# Autodesk Inventor assembly: Gripper Attempt 05
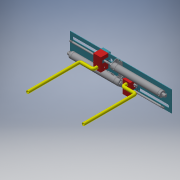
[picture p0: Inventor's stored thumbnail of the model, 180x180]
Saved by Autodesk Inventor 2016 (Build 200138000, 138)
## iProperties
Created: 2015-06-19
Part Number: Gripper Attempt 05
Document SubType Name: Assembly
Designer: steele
Mass: 1782.14 g
Surface Area: 5525.09 cm^2
Volume: 900.724 cm^3
Density: 1.97857 g/cm^3
Author: steele
## Documents named in this file (11)
- C:\snobotics\CAD-Development\robSteele\SnoBoticsSummer2015\Gripper\Gripper Attempt 05.iam
- C:\snobotics\CAD-MfgResources\McMaster-Carr\Air Cylinder\Pivot Mount Cylinders\Foot Bracket for 1_25 and 1_50 Bore\6498K340.ipt
- C:\snobotics\CAD-Development\robSteele\SnoBoticsSummer2015\Gripper\6498K681.ipt
- C:\snobotics\CAD-Development\robSteele\ipartComponents\Plate for Gripper.ipt
- C:\snobotics\CAD-Development\robSteele\SnoBoticsSummer2015\Gripper\Support For Arms.ipt
- C:\snobotics\CAD-Development\robSteele\SnoBoticsSummer2015\Gripper\Support Overlay on Gripper Side.ipt
- C:\snobotics\CAD-Development\robSteele\ipartComponents\ABS Arm.ipt
- C:\snobotics\CAD-MfgResources\McMaster-Carr\Quick Release Pin\94748A227.ipt
- C:\snobotics\autodesk\2015\FRC_FieldModel_2015\Parts\YELLOW_TOTE.ipt
- C:\snobotics\autodesk\2015\FRC_FieldModel_2015\Parts\RECYCLING_BIN_ASM.iam
- C:\snobotics\CAD-Development\robSteele\ipartComponents\Plate for Gripper\Plate for Gripper 5.5 x 27 x 1(_FS)8 x 3(_FS)8.ipt
## Components (16 placed, 9 different names)
1. Plate for Gripper 5.5 x 27 x 1(_FS)8 x 3(_FS)8:1 — Mate:1, Flush:1, Flush:2, Mate:2, Flush:3, Flush:4, Mate:9, Mate:13, Mate:14
2. 6498K340:1 — Mate:2, Flush:3, Flush:4, Mate:7
3. 6498K340:2 — Mate:1, Flush:1, Flush:2, Mate:8
4. 6498K681:1 — Mate:7
5. 6498K681:2 — Mate:8, Insert:3
6. Support For Arms:1 — Mate:9, Insert:3, Mate:10, Flush:10, Flush:13, Mate:12
7. Support For Arms:2 — Mate:13, Mate:14, Mate:15, Flush:14, Mate:16
8. Support Overlay on Gripper Side:1 — Mate:10, Flush:10, Flush:13, Mate:12, Insert:4, Insert:7
9. Support Overlay on Gripper Side:2 — Mate:15, Flush:14, Mate:16, Insert:6, Insert:8
10. ABS Arm:1 — Insert:4
11. ABS Arm:2 — Insert:6
12. 94748A227:1 — Insert:7
13. 94748A227:2 — Insert:8
14. YELLOW_TOTE:1
15. YELLOW_TOTE:2
16. RECYCLING_BIN_ASM:1 [sub-assembly]
## Relationships (23: Mate 11, Flush 7, Insert 5)
- Mate:1: Plate for Gripper 5.5 x 27 x 1(_FS)8 x 3(_FS)8:1 ↔ 6498K340:2
- Flush:1: Plate for Gripper 5.5 x 27 x 1(_FS)8 x 3(_FS)8:1 ↔ 6498K340:2
- Flush:2 (330.2 mm): Plate for Gripper 5.5 x 27 x 1(_FS)8 x 3(_FS)8:1 ↔ 6498K340:2
- Mate:2: Plate for Gripper 5.5 x 27 x 1(_FS)8 x 3(_FS)8:1 ↔ 6498K340:1
- Flush:3: Plate for Gripper 5.5 x 27 x 1(_FS)8 x 3(_FS)8:1 ↔ 6498K340:1
- Flush:4 (330.2 mm): Plate for Gripper 5.5 x 27 x 1(_FS)8 x 3(_FS)8:1 ↔ 6498K340:1
- Mate:7: 6498K340:1 ↔ 6498K681:1
- Mate:8: 6498K340:2 ↔ 6498K681:2
- Mate:9: Plate for Gripper 5.5 x 27 x 1(_FS)8 x 3(_FS)8:1 ↔ Support For Arms:1
- Insert:3: 6498K681:2 ↔ Support For Arms:1
- Mate:10: Support For Arms:1 ↔ Support Overlay on Gripper Side:1
- Flush:10: Support For Arms:1 ↔ Support Overlay on Gripper Side:1
- Flush:13: Support For Arms:1 ↔ Support Overlay on Gripper Side:1
- Mate:12: Support For Arms:1 ↔ Support Overlay on Gripper Side:1
- Insert:4 (-50.8 mm): Support Overlay on Gripper Side:1 ↔ ABS Arm:1
- Mate:13: Plate for Gripper 5.5 x 27 x 1(_FS)8 x 3(_FS)8:1 ↔ Support For Arms:2
- Mate:14: Plate for Gripper 5.5 x 27 x 1(_FS)8 x 3(_FS)8:1 ↔ Support For Arms:2
- Mate:15: Support For Arms:2 ↔ Support Overlay on Gripper Side:2
- Flush:14: Support For Arms:2 ↔ Support Overlay on Gripper Side:2
- Mate:16: Support For Arms:2 ↔ Support Overlay on Gripper Side:2
- Insert:6 (-50.8 mm): Support Overlay on Gripper Side:2 ↔ ABS Arm:2
- Insert:7: Support Overlay on Gripper Side:1 ↔ 94748A227:1
- Insert:8: Support Overlay on Gripper Side:2 ↔ 94748A227:2
## Named parameters: offsetToFrontOfAirCylinder = 330.2 mm
